# Autodesk Inventor assembly: Motor to Bearing Adapter with HSI
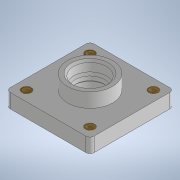
[picture p0: Inventor's stored thumbnail of the model, 180x180]
Saved by Autodesk Inventor 2022 (Build 260153000, 153)
## iProperties
Created: 2022-03-26
Part Number: Motor to Bearing Adapter with HSI
Document SubType Name: Assembly
Designer: Nick
Author: Nick
## Documents named in this file (3)
- Y:\Projects\Bibble0\3D printed\Motor to Bearing Adapter with HSI.iam
- Y:\Projects\Bibble0\3D printed\Motor to Bearing Adapter.ipt
- Y:\Projects\Bibble0\Hardware\M3 Heat Set Inserts.ipt
## Components (5 placed, 2 different names)
1. Motor to Bearing Adapter:1 — Insert:1, Insert:2, Insert:3, Insert:4
2. M3 Heat Set Inserts:1 — Insert:1
3. M3 Heat Set Inserts:2 — Insert:2
4. M3 Heat Set Inserts:3 — Insert:3
5. M3 Heat Set Inserts:4 — Insert:4
## Relationships (4: Insert 4)
- Insert:1: Motor to Bearing Adapter:1 ↔ M3 Heat Set Inserts:1
- Insert:2: Motor to Bearing Adapter:1 ↔ M3 Heat Set Inserts:2
- Insert:3: Motor to Bearing Adapter:1 ↔ M3 Heat Set Inserts:3
- Insert:4: Motor to Bearing Adapter:1 ↔ M3 Heat Set Inserts:4
